# Autodesk Inventor assembly: np2a_assembly
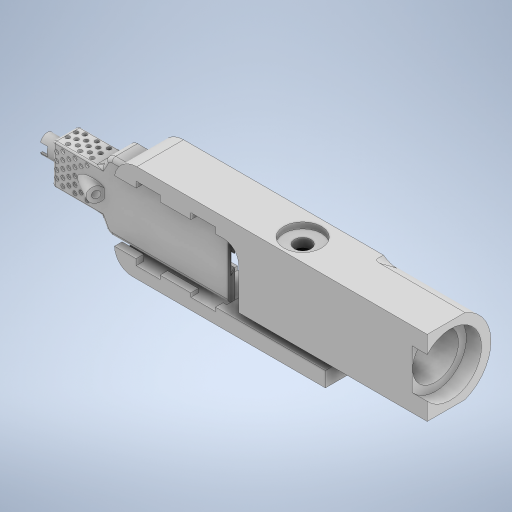
[picture p0: Inventor's stored thumbnail of the model, 512x512]
Saved by Autodesk Inventor 2023.3 (Build 273359000, 359)
## iProperties
RuleStatus: InUse
Created: 2023-07-10
Part Number: np2a_assembly
Document SubType Name: Assembly
Designer: joao
Author: joao
## Documents named in this file (7)
- X:\chronic_holder\inventor_assemblies\np2alpha_full_assembly.iam
- X:\chronic_holder\1_main_chassis\np2alpha_main_chassis.ipt
- X:\chronic_holder\2_cap\cap_no_headstage\np2alpha_cap_no_headstage.ipt
- X:\chronic_holder\3_stereotax_holder\np2alpha_stereotax_holder_part1.ipt
- X:\chronic_holder\3_stereotax_holder\np2alpha_stereotax_holder_part2.ipt
- X:\chronic_holder\2_cap\cap_with_headstage\np2alpha_cap_with_headstage.ipt
- X:\chronic_holder\2_cap\cap_with_headstage\np2alpha_headstage_cap_top_closure.ipt
## Components (6 placed, 6 different names)
1. np2alpha_main_chassis:1 — Flush:1, Flush:3, Flush:4, Flush:5, Flush:10
2. np2alpha_cap_no_headstage:1 — Flush:1, Flush:10
3. np2alpha_stereotax_holder_part1:1 — Flush:3
4. np2alpha_stereotax_holder_part2:1 — Flush:4
5. np2alpha_cap_with_headstage:1 — Flush:5, Flush:11
6. np2alpha_headstage_cap_top_closure:1 — Flush:11
## Relationships (6: Flush 6)
- Flush:1: np2alpha_main_chassis:1 ↔ np2alpha_cap_no_headstage:1
- Flush:3: np2alpha_main_chassis:1 ↔ np2alpha_stereotax_holder_part1:1
- Flush:4: np2alpha_main_chassis:1 ↔ np2alpha_stereotax_holder_part2:1
- Flush:5: np2alpha_main_chassis:1 ↔ np2alpha_cap_with_headstage:1
- Flush:10: np2alpha_main_chassis:1 ↔ np2alpha_cap_no_headstage:1
- Flush:11: np2alpha_cap_with_headstage:1 ↔ np2alpha_headstage_cap_top_closure:1
